# Autodesk Inventor assembly: YAxisMotor
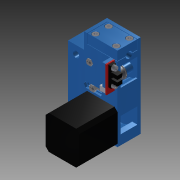
[picture p0: Inventor's stored thumbnail of the model, 180x180]
Saved by Autodesk Inventor 2015 SP1 (Build 190203100, 203)
## iProperties
Created: 2014-08-15
Part Number: YAxisMotor
Document SubType Name: Assembly
Designer: t_clevj
Mass: 238.109 g
Surface Area: 703.064 cm^2
Volume: 182.422 cm^3
Density: 1.30526 g/cm^3
Author: t_clevj
Title: Y Motor Left
## Documents named in this file (18)
- C:\Users\Jack\ownCloud\Projects\CrossBot\InventorModel\YAxis\YAxisMotorLeft.iam
- C:\Users\Jack\ownCloud\Projects\CrossBot\InventorModel\YAxis\YAxisMotor\YMotorBlockLeft.ipt
- C:\Users\Jack\ownCloud\Projects\CrossBot\InventorModel\YAxis\YAxisMotor\YMotorCapLeft.ipt
- C:\Users\Jack\ownCloud\Projects\CrossBot\InventorModel\Hardware\Bolts\SHCS\SHCS4\SHCS4x30.ipt
- C:\Users\Jack\ownCloud\Projects\CrossBot\InventorModel\Hardware\Bolts\SHCS\SHCS3\SHCS3x8.ipt
- C:\Users\Jack\ownCloud\Projects\CrossBot\InventorModel\Hardware\Bearing\BearingRadialBall\BearingRadialBallF624zz.ipt
- C:\Users\Jack\ownCloud\Projects\CrossBot\InventorModel\Hardware\Wahsers\M4Washer.ipt
- C:\Users\Jack\ownCloud\Projects\CrossBot\InventorModel\Hardware\Nuts\Nut4.ipt
- C:\Users\Jack\ownCloud\Projects\CrossBot\InventorModel\YAxis\YAxisBearingSpacer.ipt
- C:\Users\Jack\ownCloud\Projects\CrossBot\InventorModel\Electronics\Motors\StepperMotorNema17x48mm.ipt
- C:\Users\Jack\ownCloud\Projects\CrossBot\InventorModel\Hardware\Belt\GT2Idler.iam
- C:\Users\Jack\ownCloud\Projects\CrossBot\InventorModel\Hardware\Bolts\FHS\FHS4\FHS4x8.ipt
- C:\Users\Jack\ownCloud\Projects\CrossBot\InventorModel\Hardware\Bolts\SHCS\SHCS4\SHCS4x8.ipt
- C:\Users\Jack\ownCloud\Projects\CrossBot\InventorModel\YAxis\YAxisBeltIdlerSpacer.ipt
- C:\Users\Jack\ownCloud\Projects\CrossBot\InventorModel\Electronics\EndStops\EndStopOptical.ipt
- C:\Users\Jack\ownCloud\Projects\CrossBot\InventorModel\Hardware\BoltWashers\BoltWasher3\BoltWasher3x10.iam
- C:\Users\Jack\ownCloud\Projects\CrossBot\InventorModel\Hardware\Nuts\Nut3.ipt
- C:\Users\Jack\ownCloud\Projects\CrossBot\InventorModel\Hardware\Bolts\SHCS\SHCS4\SHCS4x14.ipt
## Components (44 placed, 17 different names)
1. YMotorBlockLeft:1 — Mate:4, Flush:3, Mate:5, Mate:7, Mate:8, Slider:2, Mate:9, Mate:10, Mate:11, Mate:12, Mate:13, Mate:14, Mate:15, Mate:16, Mate:17, Mate:18, Mate:30, Mate:46, Angle:1, Mate:48, Angle:2, Mate:50, Angle:3, Mate:52, Mate:82, Mate:83, Mate:84, Angle:8, Angle:9, Angle:10, Angle:11, Mate:88, Mate:89, Mate:90, Mate:91, Mate:94, Mate:99, Flush:7, Mate:100, Flush:8, Mate:101, Mate:102, Mate:103, Mate:104, Mate:106, Mate:108, Mate:109, Mate:110, Angle:12, Angle:13, Mate:117, Mate:118, Mate:120, Mate:123, Mate:124, Mate:125, Mate:126
2. YMotorCapLeft:1 — Mate:120, Mate:127, Mate:128, Mate:129, Mate:130, Mate:131, Mate:132
3. YAxisBearingSpacer:2 — Mate:77, Mate:80
4. YAxisBearingSpacer:3 — Mate:76, Mate:79
5. StepperMotorNema17x48mm:1 — Mate:82, Mate:83, Mate:84
6. GT2Idler:1 [sub-assembly] — Mate:96, Mate:121
7. YAxisBeltIdlerSpacer:1 — Mate:105, Mate:106, Mate:122
8. EndStopOptical:1 — Mate:108, Mate:109, Mate:110, Mate:111, Mate:112, Mate:113, Mate:114
9. SHCS4x14:1 — Mate:123, Mate:127, Mate:132, Mate:135
10. SHCS4x14:2 — Mate:124, Mate:128, Mate:136
11. SHCS4x14:3 — Mate:125, Mate:129, Mate:133
12. SHCS4x14:4 — Mate:126, Mate:130, Mate:131, Mate:134
13. SHCS4x30:3 — Mate:7, Mate:10, Mate:37, Mate:49, Mate:95, Mate:96, Mate:105
14. Nut4:1 — Mate:47, Angle:1, Mate:48
15. Nut4:2 — Mate:49, Angle:2, Mate:50
16. Nut4:3 — Mate:51, Angle:3, Mate:52
17. M4Washer:1 — Mate:25, Mate:26, Mate:79
18. M4Washer:2 — Mate:27, Mate:28, Mate:29, Mate:30
19. M4Washer:3 — Mate:37, Mate:121, Mate:122
20. M4Washer:4 — Mate:94, Mate:95
21. M4Washer:5 — Mate:45, Mate:80
22. M4Washer:6 — Mate:46
23. SHCS4x30:5 — Slider:2, Mate:45, Mate:51, Mate:77
24. SHCS4x30:4 — Mate:8, Mate:9, Mate:29, Mate:47, Mate:76
25. BearingRadialBallF624zz:1 — Mate:23, Mate:24, Mate:25, Mate:26
26. BearingRadialBallF624zz:6 — Mate:23, Mate:24, Mate:27, Mate:28
27. BearingRadialBallF624zz:9
28. BearingRadialBallF624zz:10
29. FHS4x8:1 — Mate:100, Flush:8
30. FHS4x8:2 — Mate:99, Flush:7
31. SHCS4x8:1 — Mate:102, Mate:103
32. SHCS4x8:2 — Mate:101, Mate:104
33. SHCS3x8:3 — Mate:14, Mate:17
34. SHCS3x8:1 — Mate:12, Mate:18
35. SHCS3x8:2 — Mate:13, Mate:16
36. SHCS3x8:4 — Mate:11, Mate:15
37. Nut4:4 — Angle:11, Mate:91, Mate:136
38. Nut4:5 — Angle:10, Mate:90, Mate:135
39. Nut4:6 — Angle:9, Mate:89, Mate:133
40. Nut4:7 — Angle:8, Mate:88, Mate:134
41. Nut3:2 — Mate:116, Angle:12, Mate:117
42. BoltWasher3x10:2 [sub-assembly] — Mate:112, Mate:114, Mate:116
43. BoltWasher3x10:1 [sub-assembly] — Mate:111, Mate:113, Mate:115
44. Nut3:1 — Mate:115, Angle:13, Mate:118
## Relationships (100: Mate 87, Angle 9, Flush 3, TranslationJoint 1)
- Mate:4: YMotorBlockLeft:1
- Flush:3: YMotorBlockLeft:1
- Mate:5: YMotorBlockLeft:1
- Mate:7: YMotorBlockLeft:1 ↔ SHCS4x30:3
- Mate:8: YMotorBlockLeft:1 ↔ SHCS4x30:4
- Slider:2 [TranslationJoint]: YMotorBlockLeft:1 ↔ SHCS4x30:5
- Mate:9: YMotorBlockLeft:1 ↔ SHCS4x30:4
- Mate:10: YMotorBlockLeft:1 ↔ SHCS4x30:3
- Mate:11: YMotorBlockLeft:1 ↔ SHCS3x8:4
- Mate:12: YMotorBlockLeft:1 ↔ SHCS3x8:1
- Mate:13: YMotorBlockLeft:1 ↔ SHCS3x8:2
- Mate:14: YMotorBlockLeft:1 ↔ SHCS3x8:3
- Mate:15: YMotorBlockLeft:1 ↔ SHCS3x8:4
- Mate:16: YMotorBlockLeft:1 ↔ SHCS3x8:2
- Mate:17: YMotorBlockLeft:1 ↔ SHCS3x8:3
- Mate:18: YMotorBlockLeft:1 ↔ SHCS3x8:1
- Mate:23: BearingRadialBallF624zz:1 ↔ BearingRadialBallF624zz:6
- Mate:24: BearingRadialBallF624zz:1 ↔ BearingRadialBallF624zz:6
- Mate:25: M4Washer:1 ↔ BearingRadialBallF624zz:1
- Mate:26: M4Washer:1 ↔ BearingRadialBallF624zz:1
- Mate:27: M4Washer:2 ↔ BearingRadialBallF624zz:6
- Mate:28: M4Washer:2 ↔ BearingRadialBallF624zz:6
- Mate:29: M4Washer:2 ↔ SHCS4x30:4
- Mate:30: YMotorBlockLeft:1 ↔ M4Washer:2
- Mate:37: SHCS4x30:3 ↔ M4Washer:3
- [Mate]: BearingRadialBallF624zz:9 ↔ BearingRadialBallF624zz:10
- [Mate]: BearingRadialBallF624zz:9 ↔ BearingRadialBallF624zz:10
- [Mate]: M4Washer:5 ↔ BearingRadialBallF624zz:9
- [Mate]: M4Washer:5 ↔ BearingRadialBallF624zz:9
- [Mate]: M4Washer:6 ↔ BearingRadialBallF624zz:10
- [Mate]: M4Washer:6 ↔ BearingRadialBallF624zz:10
- Mate:45: M4Washer:5 ↔ SHCS4x30:5
- Mate:46: YMotorBlockLeft:1 ↔ M4Washer:6
- Mate:47: Nut4:1 ↔ SHCS4x30:4
- Angle:1 (0 deg): YMotorBlockLeft:1 ↔ Nut4:1
- Mate:48: YMotorBlockLeft:1 ↔ Nut4:1
- Mate:49: SHCS4x30:3 ↔ Nut4:2
- Angle:2 (0 deg): YMotorBlockLeft:1 ↔ Nut4:2
- Mate:50: YMotorBlockLeft:1 ↔ Nut4:2
- Mate:51: Nut4:3 ↔ SHCS4x30:5
- Angle:3 (0 deg): YMotorBlockLeft:1 ↔ Nut4:3
- Mate:52: YMotorBlockLeft:1 ↔ Nut4:3
- Mate:76: YAxisBearingSpacer:3 ↔ SHCS4x30:4
- Mate:77: YAxisBearingSpacer:2 ↔ SHCS4x30:5
- Mate:79: YAxisBearingSpacer:3 ↔ M4Washer:1
- Mate:80: YAxisBearingSpacer:2 ↔ M4Washer:5
- Mate:82: YMotorBlockLeft:1 ↔ StepperMotorNema17x48mm:1
- Mate:83: YMotorBlockLeft:1 ↔ StepperMotorNema17x48mm:1
- Mate:84: YMotorBlockLeft:1 ↔ StepperMotorNema17x48mm:1
- Angle:8 (0 deg): YMotorBlockLeft:1 ↔ Nut4:7
- Angle:9 (0 deg): YMotorBlockLeft:1 ↔ Nut4:6
- Angle:10 (0 deg): YMotorBlockLeft:1 ↔ Nut4:5
- Angle:11 (0 deg): YMotorBlockLeft:1 ↔ Nut4:4
- Mate:88: YMotorBlockLeft:1 ↔ Nut4:7
- Mate:89: YMotorBlockLeft:1 ↔ Nut4:6
- Mate:90: YMotorBlockLeft:1 ↔ Nut4:5
- Mate:91: YMotorBlockLeft:1 ↔ Nut4:4
- Mate:94: YMotorBlockLeft:1 ↔ M4Washer:4
- Mate:95: SHCS4x30:3 ↔ M4Washer:4
- Mate:96: GT2Idler:1 ↔ SHCS4x30:3
- Mate:99: YMotorBlockLeft:1 ↔ FHS4x8:2
- Flush:7: YMotorBlockLeft:1 ↔ FHS4x8:2
- Mate:100: YMotorBlockLeft:1 ↔ FHS4x8:1
- Flush:8: YMotorBlockLeft:1 ↔ FHS4x8:1
- Mate:101: YMotorBlockLeft:1 ↔ SHCS4x8:2
- Mate:102: YMotorBlockLeft:1 ↔ SHCS4x8:1
- Mate:103: YMotorBlockLeft:1 ↔ SHCS4x8:1
- Mate:104: YMotorBlockLeft:1 ↔ SHCS4x8:2
- Mate:105: YAxisBeltIdlerSpacer:1 ↔ SHCS4x30:3
- Mate:106: YMotorBlockLeft:1 ↔ YAxisBeltIdlerSpacer:1
- Mate:108: YMotorBlockLeft:1 ↔ EndStopOptical:1
- Mate:109: YMotorBlockLeft:1 ↔ EndStopOptical:1
- Mate:110: YMotorBlockLeft:1 ↔ EndStopOptical:1
- Mate:111: EndStopOptical:1 ↔ BoltWasher3x10:1
- Mate:112: EndStopOptical:1 ↔ BoltWasher3x10:2
- Mate:113: EndStopOptical:1 ↔ BoltWasher3x10:1
- Mate:114: EndStopOptical:1 ↔ BoltWasher3x10:2
- Mate:115: BoltWasher3x10:1 ↔ Nut3:1
- Mate:116: Nut3:2 ↔ BoltWasher3x10:2
- Angle:12 (0 deg): YMotorBlockLeft:1 ↔ Nut3:2
- Angle:13 (0 deg): YMotorBlockLeft:1 ↔ Nut3:1
- Mate:117: YMotorBlockLeft:1 ↔ Nut3:2
- Mate:118: YMotorBlockLeft:1 ↔ Nut3:1
- Mate:120: YMotorBlockLeft:1 ↔ YMotorCapLeft:1
- Mate:121: GT2Idler:1 ↔ M4Washer:3
- Mate:122: YAxisBeltIdlerSpacer:1 ↔ M4Washer:3
- Mate:123: YMotorBlockLeft:1 ↔ SHCS4x14:1
- Mate:124: YMotorBlockLeft:1 ↔ SHCS4x14:2
- Mate:125: YMotorBlockLeft:1 ↔ SHCS4x14:3
- Mate:126: YMotorBlockLeft:1 ↔ SHCS4x14:4
- Mate:127: YMotorCapLeft:1 ↔ SHCS4x14:1
- Mate:128: YMotorCapLeft:1 ↔ SHCS4x14:2
- Mate:129: YMotorCapLeft:1 ↔ SHCS4x14:3
- Mate:130: YMotorCapLeft:1 ↔ SHCS4x14:4
- Mate:131: YMotorCapLeft:1 ↔ SHCS4x14:4
- Mate:132: YMotorCapLeft:1 ↔ SHCS4x14:1
- Mate:133: SHCS4x14:3 ↔ Nut4:6
- Mate:134: SHCS4x14:4 ↔ Nut4:7
- Mate:135: SHCS4x14:1 ↔ Nut4:5
- Mate:136: SHCS4x14:2 ↔ Nut4:4
## Named parameters: d60_d44 = 0 mm, d61_d45 = 0 mm, d62_d46 = 0 mm, d63_d47 = 0 mm, d64_d48 = 0 mm, d65_d49 = 0 mm
